# Autodesk Inventor assembly: PAM
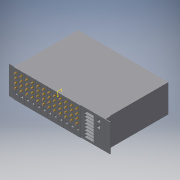
[picture p0: Inventor's stored thumbnail of the model, 180x180]
Saved by Autodesk Inventor 2016 (Build 200138000, 138)
## iProperties
Created: 2016-08-09
Part Number: PAM
Document SubType Name: Assembly
Designer: Zara
Author: Zara
## Documents named in this file (3)
- C:\Users\Zara\Documents\hera-cad\Node\PAM.iam
- C:\Users\Zara\Documents\hera-cad\Node\preamp.ipt
- C:\Users\Zara\Downloads\SMA Jack Bulkhead small nut.ipt
## Components (49 placed, 2 different names)
1. preamp:1 — Rigid:1, Rigid:2, Rigid:3, Rigid:4, Rigid:5, Rigid:6, Rigid:7, Rigid:8, Rigid:9, Rigid:10, Rigid:11, Rigid:12, Rigid:13, Rigid:14, Rigid:15, Rigid:16, Rigid:17, Rigid:18, Rigid:19, Rigid:20, Rigid:21, Rigid:22, Rigid:23, Rigid:24, Rigid:25, Rigid:26, Rigid:27, Rigid:28, Rigid:29, Rigid:30, Rigid:31, Rigid:32, Rigid:33, Rigid:34, Rigid:35, Rigid:36, Rigid:37, Rigid:38, Rigid:39, Rigid:40, Rigid:41, Rigid:42, Rigid:43, Rigid:44, Rigid:45, Rigid:46, Rigid:47, Rigid:48
2. SMA Jack Bulkhead small nut:8 — Rigid:1
3. SMA Jack Bulkhead small nut:9 — Rigid:3
4. SMA Jack Bulkhead small nut:11 — Rigid:2
5. SMA Jack Bulkhead small nut:12 — Rigid:10
6. SMA Jack Bulkhead small nut:13 — Rigid:9
7. SMA Jack Bulkhead small nut:14 — Rigid:7
8. SMA Jack Bulkhead small nut:15 — Rigid:6
9. SMA Jack Bulkhead small nut:16 — Rigid:4
10. SMA Jack Bulkhead small nut:17 — Rigid:5
11. SMA Jack Bulkhead small nut:18 — Rigid:12
12. SMA Jack Bulkhead small nut:19 — Rigid:13
13. SMA Jack Bulkhead small nut:20 — Rigid:11
14. SMA Jack Bulkhead small nut:21 — Rigid:8
15. SMA Jack Bulkhead small nut:22 — Rigid:15
16. SMA Jack Bulkhead small nut:23 — Rigid:16
17. SMA Jack Bulkhead small nut:24 — Rigid:14
18. SMA Jack Bulkhead small nut:25 — Rigid:18
19. SMA Jack Bulkhead small nut:26 — Rigid:19
20. SMA Jack Bulkhead small nut:27 — Rigid:29
21. SMA Jack Bulkhead small nut:28 — Rigid:26
22. SMA Jack Bulkhead small nut:29 — Rigid:17
23. SMA Jack Bulkhead small nut:30 — Rigid:20
24. SMA Jack Bulkhead small nut:31 — Rigid:22
25. SMA Jack Bulkhead small nut:32 — Rigid:28
26. SMA Jack Bulkhead small nut:33 — Rigid:24
27. SMA Jack Bulkhead small nut:34 — Rigid:21
28. SMA Jack Bulkhead small nut:35 — Rigid:25
29. SMA Jack Bulkhead small nut:36 — Rigid:33
30. SMA Jack Bulkhead small nut:37 — Rigid:30
31. SMA Jack Bulkhead small nut:38 — Rigid:32
32. SMA Jack Bulkhead small nut:39 — Rigid:27
33. SMA Jack Bulkhead small nut:40 — Rigid:23
34. SMA Jack Bulkhead small nut:41 — Rigid:31
35. SMA Jack Bulkhead small nut:42 — Rigid:38
36. SMA Jack Bulkhead small nut:43 — Rigid:36
37. SMA Jack Bulkhead small nut:44 — Rigid:34
38. SMA Jack Bulkhead small nut:45 — Rigid:35
39. SMA Jack Bulkhead small nut:46 — Rigid:37
40. SMA Jack Bulkhead small nut:47 — Rigid:39
41. SMA Jack Bulkhead small nut:48 — Rigid:40
42. SMA Jack Bulkhead small nut:49 — Rigid:44
43. SMA Jack Bulkhead small nut:50 — Rigid:43
44. SMA Jack Bulkhead small nut:51 — Rigid:42
45. SMA Jack Bulkhead small nut:52 — Rigid:45
46. SMA Jack Bulkhead small nut:53 — Rigid:46
47. SMA Jack Bulkhead small nut:54 — Rigid:41
48. SMA Jack Bulkhead small nut:55 — Rigid:47
49. SMA Jack Bulkhead small nut:56 — Rigid:48
## Relationships (48: WeldJoint 48)
- Rigid:1 [WeldJoint]: preamp:1 ↔ SMA Jack Bulkhead small nut:8
- Rigid:2 [WeldJoint]: preamp:1 ↔ SMA Jack Bulkhead small nut:11
- Rigid:3 [WeldJoint]: preamp:1 ↔ SMA Jack Bulkhead small nut:9
- Rigid:4 [WeldJoint]: preamp:1 ↔ SMA Jack Bulkhead small nut:16
- Rigid:5 [WeldJoint]: preamp:1 ↔ SMA Jack Bulkhead small nut:17
- Rigid:6 [WeldJoint]: preamp:1 ↔ SMA Jack Bulkhead small nut:15
- Rigid:7 [WeldJoint]: preamp:1 ↔ SMA Jack Bulkhead small nut:14
- Rigid:8 [WeldJoint]: preamp:1 ↔ SMA Jack Bulkhead small nut:21
- Rigid:9 [WeldJoint]: preamp:1 ↔ SMA Jack Bulkhead small nut:13
- Rigid:10 [WeldJoint]: preamp:1 ↔ SMA Jack Bulkhead small nut:12
- Rigid:11 [WeldJoint]: preamp:1 ↔ SMA Jack Bulkhead small nut:20
- Rigid:12 [WeldJoint]: preamp:1 ↔ SMA Jack Bulkhead small nut:18
- Rigid:13 [WeldJoint]: preamp:1 ↔ SMA Jack Bulkhead small nut:19
- Rigid:14 [WeldJoint]: preamp:1 ↔ SMA Jack Bulkhead small nut:24
- Rigid:15 [WeldJoint]: preamp:1 ↔ SMA Jack Bulkhead small nut:22
- Rigid:16 [WeldJoint]: preamp:1 ↔ SMA Jack Bulkhead small nut:23
- Rigid:17 [WeldJoint]: preamp:1 ↔ SMA Jack Bulkhead small nut:29
- Rigid:18 [WeldJoint]: preamp:1 ↔ SMA Jack Bulkhead small nut:25
- Rigid:19 [WeldJoint]: preamp:1 ↔ SMA Jack Bulkhead small nut:26
- Rigid:20 [WeldJoint]: preamp:1 ↔ SMA Jack Bulkhead small nut:30
- Rigid:21 [WeldJoint]: preamp:1 ↔ SMA Jack Bulkhead small nut:34
- Rigid:22 [WeldJoint]: preamp:1 ↔ SMA Jack Bulkhead small nut:31
- Rigid:23 [WeldJoint]: preamp:1 ↔ SMA Jack Bulkhead small nut:40
- Rigid:24 [WeldJoint]: preamp:1 ↔ SMA Jack Bulkhead small nut:33
- Rigid:25 [WeldJoint]: preamp:1 ↔ SMA Jack Bulkhead small nut:35
- Rigid:26 [WeldJoint]: preamp:1 ↔ SMA Jack Bulkhead small nut:28
- Rigid:27 [WeldJoint]: preamp:1 ↔ SMA Jack Bulkhead small nut:39
- Rigid:28 [WeldJoint]: preamp:1 ↔ SMA Jack Bulkhead small nut:32
- Rigid:29 [WeldJoint]: preamp:1 ↔ SMA Jack Bulkhead small nut:27
- Rigid:30 [WeldJoint]: preamp:1 ↔ SMA Jack Bulkhead small nut:37
- Rigid:31 [WeldJoint]: preamp:1 ↔ SMA Jack Bulkhead small nut:41
- Rigid:32 [WeldJoint]: preamp:1 ↔ SMA Jack Bulkhead small nut:38
- Rigid:33 [WeldJoint]: preamp:1 ↔ SMA Jack Bulkhead small nut:36
- Rigid:34 [WeldJoint]: preamp:1 ↔ SMA Jack Bulkhead small nut:44
- Rigid:35 [WeldJoint]: preamp:1 ↔ SMA Jack Bulkhead small nut:45
- Rigid:36 [WeldJoint]: preamp:1 ↔ SMA Jack Bulkhead small nut:43
- Rigid:37 [WeldJoint]: preamp:1 ↔ SMA Jack Bulkhead small nut:46
- Rigid:38 [WeldJoint]: preamp:1 ↔ SMA Jack Bulkhead small nut:42
- Rigid:39 [WeldJoint]: preamp:1 ↔ SMA Jack Bulkhead small nut:47
- Rigid:40 [WeldJoint]: preamp:1 ↔ SMA Jack Bulkhead small nut:48
- Rigid:41 [WeldJoint]: preamp:1 ↔ SMA Jack Bulkhead small nut:54
- Rigid:42 [WeldJoint]: preamp:1 ↔ SMA Jack Bulkhead small nut:51
- Rigid:43 [WeldJoint]: preamp:1 ↔ SMA Jack Bulkhead small nut:50
- Rigid:44 [WeldJoint]: preamp:1 ↔ SMA Jack Bulkhead small nut:49
- Rigid:45 [WeldJoint]: preamp:1 ↔ SMA Jack Bulkhead small nut:52
- Rigid:46 [WeldJoint]: preamp:1 ↔ SMA Jack Bulkhead small nut:53
- Rigid:47 [WeldJoint]: preamp:1 ↔ SMA Jack Bulkhead small nut:55
- Rigid:48 [WeldJoint]: preamp:1 ↔ SMA Jack Bulkhead small nut:56
